# Autodesk Inventor assembly: Torre
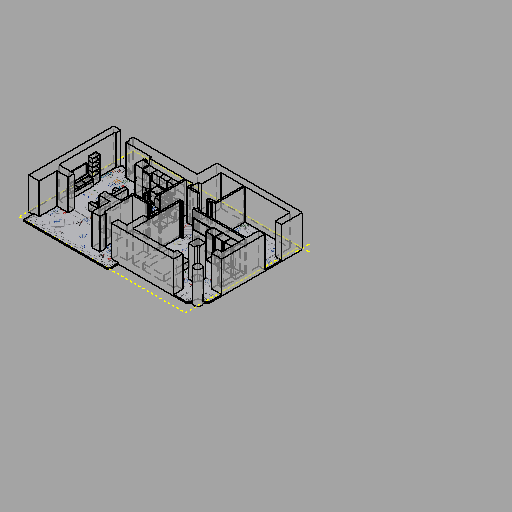
[picture p0: Inventor's stored thumbnail of the model, 512x512]
Saved by Autodesk Inventor 2025.2 (Build 292293000, 293)
## iProperties
Created: 2025-08-11
Part Number: Torre
Document SubType Name: Assembly
Designer: Luca
Mass: 7.82571e+07 g
Surface Area: 6.47203e+06 cm^2
Volume: 7.82582e+07 cm^3
Density: 0.999986 g/cm^3
FORNITO DA: ###
Author: Luca
## Documents named in this file (14)
- C:\Users\tecnico11\Desktop\Luca\Torre\Torre.iam
- C:\Users\tecnico11\Desktop\Luca\Torre\Planimetria.ipt
- C:\Users\tecnico11\Desktop\Luca\Torre\PAX.ipt
- C:\Users\tecnico11\Desktop\Luca\Torre\TV 65.ipt
- C:\Users\tecnico11\Desktop\Luca\Torre\Letto generico.ipt
- C:\Users\tecnico11\Desktop\Luca\Torre\Mobile TV.ipt
- C:\Users\tecnico11\Desktop\Luca\Torre\Libreria.ipt
- C:\Users\tecnico11\Desktop\Luca\Torre\Divano.ipt
- C:\Users\tecnico11\Desktop\Luca\Torre\Top cucina.ipt
- C:\Users\tecnico11\Desktop\Luca\Torre\Microonde.ipt
- C:\Users\tecnico11\Desktop\Luca\Torre\Divano Valdinoce.ipt
- C:\Users\tecnico11\Desktop\Luca\Torre\Cucina.iam
- C:\Users\tecnico11\Desktop\Luca\Torre\Mobiletto verticale.ipt
- C:\Users\tecnico11\Desktop\Luca\Torre\Tecnico 3D.ipt
## Components (18 placed, 13 different names)
1. Planimetria:1 — Coincidente:1, Coincidente:3, Coincidente:4, Coincidente:7, Coincidente:8, Coincidente:14, Coincidente:15, Allineato:17, Coincidente:17, Coincidente:18, Coincidente:19, Coincidente:20, Coincidente:21, Coincidente:22, Coincidente:23, Coincidente:24, Coincidente:25, Coincidente:26, Coincidente:28, Allineato:19, Coincidente:54, Allineato:20, Coincidente:66
2. PAX:1 — Coincidente:1, Coincidente:3, Coincidente:5, Coincidente:6
3. PAX:3 — Coincidente:5, Coincidente:6, Coincidente:8, Coincidente:9
4. PAX:2 — Coincidente:4, Coincidente:7, Coincidente:9, Coincidente:10, Coincidente:13
5. PAX:4 — Coincidente:10, Coincidente:11, Coincidente:12, Coincidente:13
6. PAX:5 — Coincidente:11, Coincidente:12
7. TV 65:1 — Coincidente:14, Coincidente:15, Allineato:17
8. Letto generico:1 — Coincidente:17, Coincidente:18, Coincidente:19
9. TV 65:2 — Coincidente:20, Coincidente:21, Allineato:18, Coincidente:55
10. Mobile TV:1 — Coincidente:22, Coincidente:23, Allineato:18, Coincidente:24, Coincidente:27, Coincidente:29
11. Libreria:1 — Coincidente:25, Coincidente:26, Coincidente:27
12. Divano:1 — Coincidente:28, Coincidente:29, Allineato:19
13. Top cucina:1 — Coincidente:45
14. Microonde:1 — Coincidente:45
15. Divano Valdinoce:1 — Coincidente:54, Allineato:20, Coincidente:55
16. Cucina:1 [sub-assembly] — Coincidente:64, Coincidente:65
17. Mobiletto verticale:1 — Coincidente:64, Coincidente:65
18. Tecnico 3D:1 — Coincidente:66
## Relationships (42: Mate 37, Flush 4, WeldJoint 1)
- Coincidente:1 [Mate]: Planimetria:1 ↔ PAX:1
- Coincidente:3 [Mate]: Planimetria:1 ↔ PAX:1
- Coincidente:4 [Mate]: Planimetria:1 ↔ PAX:2
- Coincidente:5 [Mate]: PAX:1 ↔ PAX:3
- Coincidente:6 [Mate]: PAX:1 ↔ PAX:3
- Coincidente:7 [Mate]: Planimetria:1 ↔ PAX:2
- Coincidente:8 [Mate]: Planimetria:1 ↔ PAX:3
- Coincidente:9 [Mate]: PAX:3 ↔ PAX:2
- Coincidente:10 [Mate]: PAX:2 ↔ PAX:4
- Coincidente:11 [Mate]: PAX:4 ↔ PAX:5
- Coincidente:12 [Mate]: PAX:4 ↔ PAX:5
- Coincidente:13 [Mate]: PAX:2 ↔ PAX:4
- Coincidente:14 [Mate]: Planimetria:1 ↔ TV 65:1
- Coincidente:15 [Mate] (1100 mm): Planimetria:1 ↔ TV 65:1
- Allineato:17 [Flush] (-100 mm): Planimetria:1 ↔ TV 65:1
- Coincidente:17 [Mate]: Planimetria:1 ↔ Letto generico:1
- Coincidente:18 [Mate]: Planimetria:1 ↔ Letto generico:1
- Coincidente:19 [Mate] (1650 mm): Planimetria:1 ↔ Letto generico:1
- Coincidente:20 [Mate]: Planimetria:1 ↔ TV 65:2
- Coincidente:21 [Mate] (750 mm): Planimetria:1 ↔ TV 65:2
- Coincidente:22 [Mate]: Planimetria:1 ↔ Mobile TV:1
- Coincidente:23 [Mate]: Planimetria:1 ↔ Mobile TV:1
- Allineato:18 [Flush]: TV 65:2 ↔ Mobile TV:1
- Coincidente:24 [Mate] (600 mm): Planimetria:1 ↔ Mobile TV:1
- Coincidente:25 [Mate]: Planimetria:1 ↔ Libreria:1
- Coincidente:26 [Mate]: Planimetria:1 ↔ Libreria:1
- Coincidente:27 [Mate]: Mobile TV:1 ↔ Libreria:1
- Coincidente:28 [Mate]: Planimetria:1 ↔ Divano:1
- Coincidente:29 [Mate]: Mobile TV:1 ↔ Divano:1
- Allineato:19 [Flush] (3000 mm): Planimetria:1 ↔ Divano:1
- Coincidente:45 [Mate]: Top cucina:1 ↔ Microonde:1
- [Mate] (50 mm): Microonde:1 ↔ Cucina:1
- [Mate]: Planimetria:1 ↔ Cucina:1
- [Mate]: Planimetria:1 ↔ Cucina:1
- [WeldJoint]: Top cucina:1 ↔ Cucina:1
- Coincidente:54 [Mate]: Planimetria:1 ↔ Divano Valdinoce:1
- Allineato:20 [Flush] (-3000 mm): Planimetria:1 ↔ Divano Valdinoce:1
- Coincidente:55 [Mate]: TV 65:2 ↔ Divano Valdinoce:1
- [Mate]: Planimetria:1 ↔ Cucina:1
- Coincidente:64 [Mate]: Cucina:1 ↔ Mobiletto verticale:1
- Coincidente:65 [Mate]: Cucina:1 ↔ Mobiletto verticale:1
- Coincidente:66 [Mate]: Planimetria:1 ↔ Tecnico 3D:1
